# Autodesk Inventor assembly: R-SO v11
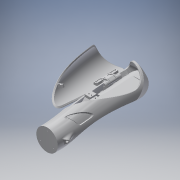
[picture p0: Inventor's stored thumbnail of the model, 180x180]
Saved by Autodesk Inventor 2018.2 (Build 222227000, 227)
## iProperties
Created: 2017-09-22
Part Number: R-SO v11
Material: 一般
Document SubType Name: Assembly
Designer: sktom
Author: sktom
## Documents named in this file (10)
- D:\CloudStrage\OneDrive\CADMech\HbSizeMMech\UnitSocket\Unit_MR-SO.iam
- D:\CloudStrage\OneDrive\CADMech\HbSizeMMech\UnitSocket\MR-SO-02.ipt
- D:\CloudStrage\OneDrive\CADMech\HbSizeMMech\UnitSocket\MR-SO-01.ipt
- D:\CloudStrage\OneDrive\CADMech\HbSizeMMech\UnitSocket\MR-SO-05.ipt
- D:\CloudStrage\OneDrive\CADMech\HbSizeMMech\UnitSocket\MR-SO-06.ipt
- D:\CloudStrage\OneDrive\CADMech\HbSizeMMech\UnitSocket\MR-SO-07.ipt
- D:\CloudStrage\OneDrive\CADMech\HbSizeMMech\UnitSocket\MR-SO-08.ipt
- D:\CloudStrage\OneDrive\CADMech\HbSizeMMech\UnitSocket\MR-SO-09.ipt
- D:\CloudStrage\OneDrive\CADMech\HbSizeMMech\UnitSocket\MR-SO-10.ipt
- D:\CloudStrage\OneDrive\CADMech\HbSizeMMech\UnitSocket\Parts_Screw_M2_L8.ipt
## Components (15 placed, 9 different names)
1. R-SO-01 v2:1 — リジッド:2, 挿入:7, 挿入:11, 挿入:12
2. R-SO-02 v2:1 — リジッド:2, メイト:1, メイト:2, 挿入:9, 挿入:10, 挿入:13, 挿入:14
3. R-SO-05 v2:1 — メイト:1, メイト:2, メイト:3, メイト:4, メイト:5
4. R-SO-06 v2:1 — メイト:3, メイト:4, メイト:5, 挿入:8
5. R-SO-07 v2:1 — 挿入:1, 挿入:2, 挿入:3, 挿入:4, 挿入:5, 挿入:6, 挿入:7
6. R-SO-08 v2:1 — 挿入:5, 挿入:6
7. R-SO-09 v2:1 — 挿入:1, 挿入:2
8. R-SO-10 v2:1 — 挿入:3, 挿入:4
9. Parts_Screw_M2_L8:1 — 挿入:8
10. Parts_Screw_M2_L8:2 — 挿入:11
11. Parts_Screw_M2_L8:3 — 挿入:9
12. Parts_Screw_M2_L8:4 — 挿入:14
13. Parts_Screw_M2_L8:5 — 挿入:13
14. Parts_Screw_M2_L8:6 — 挿入:10
15. Parts_Screw_M2_L8:7 — 挿入:12
## Relationships (20: Insert 14, Mate 5, WeldJoint 1)
- リジッド:2 [WeldJoint] (-0.14 mm): R-SO-01 v2:1 ↔ R-SO-02 v2:1
- 挿入:1 [Insert]: R-SO-07 v2:1 ↔ R-SO-09 v2:1
- 挿入:2 [Insert]: R-SO-07 v2:1 ↔ R-SO-09 v2:1
- 挿入:3 [Insert]: R-SO-07 v2:1 ↔ R-SO-10 v2:1
- 挿入:4 [Insert]: R-SO-07 v2:1 ↔ R-SO-10 v2:1
- 挿入:5 [Insert]: R-SO-07 v2:1 ↔ R-SO-08 v2:1
- 挿入:6 [Insert]: R-SO-07 v2:1 ↔ R-SO-08 v2:1
- 挿入:7 [Insert] (0.2 mm): R-SO-01 v2:1 ↔ R-SO-07 v2:1
- メイト:1 [Mate] (0.1 mm): R-SO-02 v2:1 ↔ R-SO-05 v2:1
- メイト:2 [Mate] (0.1 mm): R-SO-02 v2:1 ↔ R-SO-05 v2:1
- メイト:3 [Mate]: R-SO-05 v2:1 ↔ R-SO-06 v2:1
- メイト:4 [Mate]: R-SO-05 v2:1 ↔ R-SO-06 v2:1
- メイト:5 [Mate]: R-SO-05 v2:1 ↔ R-SO-06 v2:1
- 挿入:8 [Insert]: R-SO-06 v2:1 ↔ Parts_Screw_M2_L8:1
- 挿入:9 [Insert]: R-SO-02 v2:1 ↔ Parts_Screw_M2_L8:3
- 挿入:10 [Insert]: R-SO-02 v2:1 ↔ Parts_Screw_M2_L8:6
- 挿入:11 [Insert]: R-SO-01 v2:1 ↔ Parts_Screw_M2_L8:2
- 挿入:12 [Insert]: R-SO-01 v2:1 ↔ Parts_Screw_M2_L8:7
- 挿入:13 [Insert]: R-SO-02 v2:1 ↔ Parts_Screw_M2_L8:5
- 挿入:14 [Insert]: R-SO-02 v2:1 ↔ Parts_Screw_M2_L8:4
